# Autodesk Inventor assembly: COTS_PA-01
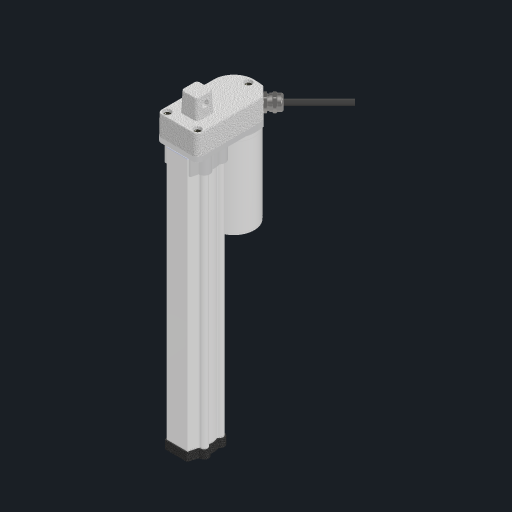
[picture p0: Inventor's stored thumbnail of the model, 512x512]
Saved by Autodesk Inventor 2024.2 (Build 282272000, 272)
## iProperties
Created: 2024-11-28
Part Number: COTS_PA-01
Document SubType Name: Assembly
Designer: Bryan
Mass: 1154.28 g
Surface Area: 870.431 cm^2
Volume: 383.444 cm^3
Density: 3.0103 g/cm^3
Author: Bryan
## Documents named in this file (18)
- C:\Users\bobsb\OneDrive\Documents\GitHub\1622-2024-Casino-Clash-CAD-A-Thon\COTS Library\Motion\Linear Actuators\PA-01\COTS_PA-01.iam
- C:\Users\bobsb\OneDrive\Documents\GitHub\1622-2024-Casino-Clash-CAD-A-Thon\COTS Library\Motion\Linear Actuators\PA-01\Solid7.ipt
- C:\Users\bobsb\OneDrive\Documents\GitHub\1622-2024-Casino-Clash-CAD-A-Thon\COTS Library\Motion\Linear Actuators\PA-01\Solid5.ipt
- C:\Users\bobsb\OneDrive\Documents\GitHub\1622-2024-Casino-Clash-CAD-A-Thon\COTS Library\Motion\Linear Actuators\PA-01\Solid1.ipt
- C:\Users\bobsb\OneDrive\Documents\GitHub\1622-2024-Casino-Clash-CAD-A-Thon\COTS Library\Motion\Linear Actuators\PA-01\Solid2.ipt
- C:\Users\bobsb\OneDrive\Documents\GitHub\1622-2024-Casino-Clash-CAD-A-Thon\COTS Library\Motion\Linear Actuators\PA-01\Solid3.ipt
- C:\Users\bobsb\OneDrive\Documents\GitHub\1622-2024-Casino-Clash-CAD-A-Thon\COTS Library\Motion\Linear Actuators\PA-01\Solid4.ipt
- C:\Users\bobsb\OneDrive\Documents\GitHub\1622-2024-Casino-Clash-CAD-A-Thon\COTS Library\Motion\Linear Actuators\PA-01\Solid6.ipt
- C:\Users\bobsb\OneDrive\Documents\GitHub\1622-2024-Casino-Clash-CAD-A-Thon\COTS Library\Motion\Linear Actuators\PA-01\Solid8.ipt
- C:\Users\bobsb\OneDrive\Documents\GitHub\1622-2024-Casino-Clash-CAD-A-Thon\COTS Library\Motion\Linear Actuators\PA-01\Solid9.ipt
- C:\Users\bobsb\OneDrive\Documents\GitHub\1622-2024-Casino-Clash-CAD-A-Thon\COTS Library\Motion\Linear Actuators\PA-01\Solid10.ipt
- C:\Users\bobsb\OneDrive\Documents\GitHub\1622-2024-Casino-Clash-CAD-A-Thon\COTS Library\Motion\Linear Actuators\PA-01\Solid11.ipt
- C:\Users\bobsb\OneDrive\Documents\GitHub\1622-2024-Casino-Clash-CAD-A-Thon\COTS Library\Motion\Linear Actuators\PA-01\Solid12.ipt
- C:\Users\bobsb\OneDrive\Documents\GitHub\1622-2024-Casino-Clash-CAD-A-Thon\COTS Library\Motion\Linear Actuators\PA-01\Solid13.ipt
- C:\Users\bobsb\OneDrive\Documents\GitHub\1622-2024-Casino-Clash-CAD-A-Thon\COTS Library\Motion\Linear Actuators\PA-01\Solid14.ipt
- C:\Users\bobsb\OneDrive\Documents\GitHub\1622-2024-Casino-Clash-CAD-A-Thon\COTS Library\Motion\Linear Actuators\PA-01\Solid15.ipt
- C:\Users\bobsb\OneDrive\Documents\GitHub\1622-2024-Casino-Clash-CAD-A-Thon\COTS Library\Motion\Linear Actuators\PA-01\Solid16.ipt
- C:\Users\bobsb\OneDrive\Documents\GitHub\1622-2024-Casino-Clash-CAD-A-Thon\COTS Library\Motion\Linear Actuators\PA-01\Solid17.ipt
## Components (17 placed, 17 different names)
1. Solid7:1 — Mate:20
2. Solid5:1 — Mate:2, Mate:3, Mate:18, Mate:19
3. Solid1:1
4. Solid2:1
5. Solid3:1 — Mate:2, Mate:3
6. Solid4:1
7. Solid6:1
8. Solid8:1 — Mate:15, Mate:16, Mate:17, Mate:18, Mate:19
9. Solid9:1 — Mate:4, Mate:5, Mate:6, Mate:7, Mate:8, Mate:9, Mate:10, Mate:11, Mate:12, Mate:13, Mate:14, Mate:15, Mate:16, Mate:17, Mate:20
10. Solid10:1 — Mate:12, Mate:13, Mate:14
11. Solid11:1 — Mate:6, Mate:8
12. Solid12:1 — Mate:4, Mate:10
13. Solid13:1 — Mate:7, Mate:9
14. Solid14:1 — Mate:5, Mate:11
15. Solid15:1
16. Solid16:1
17. Solid17:1
## Relationships (19: Mate 19)
- Mate:2: Solid5:1 ↔ Solid3:1
- Mate:3: Solid5:1 ↔ Solid3:1
- Mate:4: Solid9:1 ↔ Solid12:1
- Mate:5: Solid9:1 ↔ Solid14:1
- Mate:6: Solid9:1 ↔ Solid11:1
- Mate:7: Solid9:1 ↔ Solid13:1
- Mate:8: Solid9:1 ↔ Solid11:1
- Mate:9: Solid9:1 ↔ Solid13:1
- Mate:10: Solid9:1 ↔ Solid12:1
- Mate:11: Solid9:1 ↔ Solid14:1
- Mate:12: Solid9:1 ↔ Solid10:1
- Mate:13: Solid9:1 ↔ Solid10:1
- Mate:14: Solid9:1 ↔ Solid10:1
- Mate:15: Solid8:1 ↔ Solid9:1
- Mate:16: Solid8:1 ↔ Solid9:1
- Mate:17 (0.6 mm): Solid8:1 ↔ Solid9:1
- Mate:18: Solid5:1 ↔ Solid8:1
- Mate:19: Solid5:1 ↔ Solid8:1
- Mate:20 (-295.962 mm): Solid7:1 ↔ Solid9:1
